# Autodesk Inventor assembly: hatch above arm
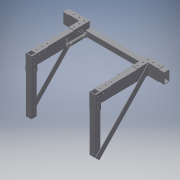
[picture p0: Inventor's stored thumbnail of the model, 180x180]
Saved by Autodesk Inventor 2018 (Build 220112000, 112)
## iProperties
Created: 2019-01-20
Part Number: hatch above arm
Document SubType Name: Assembly
Designer: Burni
Author: Burni
## Documents named in this file (7)
- C:\Users\Burni\Desktop\Robotics\final Hatch design\hatch above arm.iam
- C:\Users\Burni\Desktop\Robotics\final Hatch design\left arm.ipt
- C:\Users\Burni\Desktop\Robotics\final Hatch design\right arm.ipt
- C:\Users\Burni\Desktop\Robotics\final Hatch design\push bar.ipt
- C:\Users\Burni\Desktop\Robotics\final Hatch design\PARTserver02019011803125824465437192d056f\AIS2018\021-DXP(F,D-770).iam
- C:\Users\Burni\Desktop\Robotics\final Hatch design\Bracing 3x3.ipt
- C:\Users\Burni\OneDrive\Documents\supports.ipt
## Components (17 placed, 6 different names)
1. left arm:1 — Mate:20, Flush:20, Mate:26, Flush:26, Flush:27
2. right arm:1 — Mate:21, Flush:21, Mate:22, Flush:25, Mate:31
3. push bar:1
4. 021-DXP(F,D-770):1 [sub-assembly]
5. 021-DXP(F,D-770):2 [sub-assembly]
6. Bracing 3x3:1 — Mate:29
7. Bracing 3x3:2
8. Bracing 3x3:3
9. Bracing 3x3:4 — Mate:33
10. Bracing 3x3:5 — Mate:24, Flush:24, Flush:25
11. Bracing 3x3:6 — Mate:20, Flush:20, Flush:28
12. Bracing 3x3:7 — Mate:21, Flush:21, Mate:22, Mate:23, Flush:22, Flush:23
13. Bracing 3x3:8 — Flush:29, Flush:30, Mate:27
14. push bar:2 — Mate:26, Flush:26, Flush:27, Flush:28, Flush:29, Flush:30, Mate:27, Flush:31, Mate:28, Mate:30
15. push bar:3 — Mate:23, Flush:22, Flush:23, Mate:24, Flush:24, Mate:32
16. supports:1 — Flush:31, Mate:28, Mate:29, Mate:30
17. supports:4 — Mate:31, Mate:32, Mate:33
## Relationships (47: Mate 24, Flush 23)
- [Mate]: left arm:1 ↔ 021-DXP(F,D-770):1
- [Mate]: right arm:1 ↔ 021-DXP(F,D-770):2
- [Flush]: right arm:1 ↔ Bracing 3x3:4
- [Flush]: right arm:1 ↔ Bracing 3x3:4
- [Mate]: right arm:1 ↔ Bracing 3x3:4
- [Flush]: right arm:1 ↔ Bracing 3x3:3
- [Mate]: right arm:1 ↔ Bracing 3x3:3
- [Flush]: right arm:1 ↔ Bracing 3x3:3
- [Flush]: left arm:1 ↔ Bracing 3x3:1
- [Flush]: left arm:1 ↔ Bracing 3x3:1
- [Mate]: left arm:1 ↔ Bracing 3x3:1
- [Mate]: left arm:1 ↔ Bracing 3x3:2
- [Flush]: left arm:1 ↔ Bracing 3x3:2
- [Flush]: left arm:1 ↔ Bracing 3x3:2
- [Flush]: left arm:1 ↔ right arm:1
- [Mate] (2.54 mm): push bar:1 ↔ 021-DXP(F,D-770):2
- [Mate] (279.4 mm): left arm:1 ↔ right arm:1
- [Mate]: push bar:1 ↔ 021-DXP(F,D-770):2
- [Mate] (2.54 mm): push bar:1 ↔ 021-DXP(F,D-770):1
- [Mate]: push bar:1 ↔ 021-DXP(F,D-770):1
- [Flush] (38.1 mm): right arm:1 ↔ 021-DXP(F,D-770):2
- [Flush] (38.1 mm): left arm:1 ↔ 021-DXP(F,D-770):1
- Mate:20: left arm:1 ↔ Bracing 3x3:6
- Flush:20: left arm:1 ↔ Bracing 3x3:6
- Mate:21: right arm:1 ↔ Bracing 3x3:7
- Flush:21: right arm:1 ↔ Bracing 3x3:7
- Mate:22: right arm:1 ↔ Bracing 3x3:7
- Mate:23: Bracing 3x3:7 ↔ push bar:3
- Flush:22: Bracing 3x3:7 ↔ push bar:3
- Flush:23: Bracing 3x3:7 ↔ push bar:3
- Mate:24: Bracing 3x3:5 ↔ push bar:3
- Flush:24: Bracing 3x3:5 ↔ push bar:3
- Flush:25: right arm:1 ↔ Bracing 3x3:5
- Mate:26: left arm:1 ↔ push bar:2
- Flush:26: left arm:1 ↔ push bar:2
- Flush:27: left arm:1 ↔ push bar:2
- Flush:28: Bracing 3x3:6 ↔ push bar:2
- Flush:29: Bracing 3x3:8 ↔ push bar:2
- Flush:30: Bracing 3x3:8 ↔ push bar:2
- Mate:27: Bracing 3x3:8 ↔ push bar:2
- Flush:31: push bar:2 ↔ supports:1
- Mate:28: push bar:2 ↔ supports:1
- Mate:29: Bracing 3x3:1 ↔ supports:1
- Mate:30: push bar:2 ↔ supports:1
- Mate:31: right arm:1 ↔ supports:4
- Mate:32: push bar:3 ↔ supports:4
- Mate:33: Bracing 3x3:4 ↔ supports:4
## Named parameters: d9_d32 = 0 mm
